# Autodesk Inventor assembly: KS-14_SLow_kaiseki
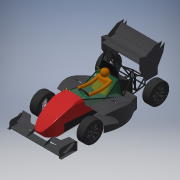
[picture p0: Inventor's stored thumbnail of the model, 180x180]
Saved by Autodesk Inventor 2018.2 (Build 222227000, 227)
## iProperties
Created: 2017-11-01
Part Number: KS-14_SLow_kaiseki
Material: 一般
Document SubType Name: Assembly
Designer: kuwano
Author: kuwano
## Documents named in this file (8)
- Z:\各班フォルダ\2018\ボディ\カウル\AeroCAD2018\CAD\Inventor\解析用CAD\KS-14_SLow_kaiseki.iam
- Z:\各班フォルダ\2018\ボディ\カウル\AeroCAD2018\CAD\Inventor\Assembly(KS-14.ver)\KS-14_SLow\KS-14_SLow.iam
- Z:\各班フォルダ\2018\ボディ\カウル\AeroCAD2018\CAD\Inventor\解析用CAD\R-wing\Rwing.iam
- Z:\各班フォルダ\2018\ボディ\カウル\AeroCAD2018\CAD\Inventor\Aero Parts\F-wing\type7\F-wing.iam
- Z:\各班フォルダ\2018\ボディ\カウル\AeroCAD2018\CAD\Inventor\Aero Parts\Side Pontoon\type3(kuwano)\defuser.ipt
- Z:\各班フォルダ\2018\ボディ\カウル\AeroCAD2018\CAD\Inventor\Aero Parts\Side Pontoon\type3(kuwano)\defuser_MIR.ipt
- Z:\各班フォルダ\2018\ボディ\カウル\AeroCAD2018\CAD\Inventor\Aero Parts\Side Pontoon\type3(kuwano)\test.ipt
- Z:\各班フォルダ\2018\ボディ\カウル\AeroCAD2018\CAD\Inventor\Aero Parts\Side Pontoon\type3(kuwano)\test_MIR.ipt
## Components (7 placed, 7 different names)
1. KS-14_SLow:1 [sub-assembly] — メイト:1, フラッシュ:1, 正接:1, 角度:1
2. Rwing:1 [sub-assembly] — フラッシュ:2, 角度:1
3. F-wing:1 [sub-assembly] — フラッシュ:3
4. defuser:1 — メイト:2, メイト:3, メイト:4
5. defuser_MIR:1 — メイト:5, メイト:6, メイト:7
6. test:1 — メイト:2, メイト:3, メイト:4, メイト:8, メイト:9, メイト:10, メイト:11
7. test_MIR:1 — メイト:5, メイト:6, メイト:7, メイト:8, メイト:9, メイト:10
## Relationships (16: Mate 11, Flush 3, Tangent 1, Angle 1)
- メイト:1 [Mate]: KS-14_SLow:1
- フラッシュ:1 [Flush]: KS-14_SLow:1
- 正接:1 [Tangent]: KS-14_SLow:1
- フラッシュ:2 [Flush]: Rwing:1
- 角度:1 [Angle] (0 deg): KS-14_SLow:1 ↔ Rwing:1
- フラッシュ:3 [Flush]: F-wing:1
- メイト:2 [Mate]: defuser:1 ↔ test:1
- メイト:3 [Mate]: defuser:1 ↔ test:1
- メイト:4 [Mate]: defuser:1 ↔ test:1
- メイト:5 [Mate]: defuser_MIR:1 ↔ test_MIR:1
- メイト:6 [Mate]: defuser_MIR:1 ↔ test_MIR:1
- メイト:7 [Mate]: defuser_MIR:1 ↔ test_MIR:1
- メイト:8 [Mate]: test:1 ↔ test_MIR:1
- メイト:9 [Mate]: test:1 ↔ test_MIR:1
- メイト:10 [Mate]: test:1 ↔ test_MIR:1
- メイト:11 [Mate]: test:1
